# Autodesk Inventor assembly: VerticalSlides2.1
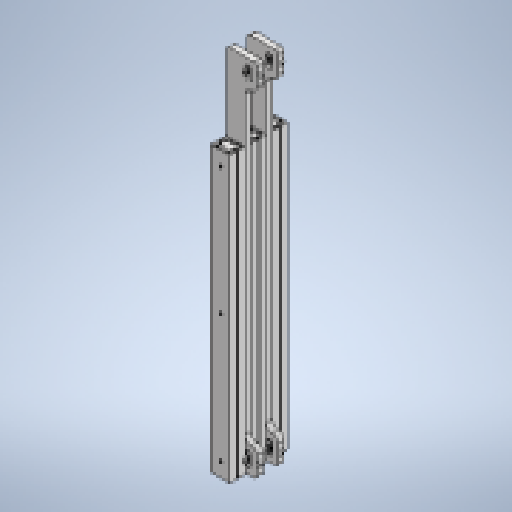
[picture p0: Inventor's stored thumbnail of the model, 512x512]
Saved by Autodesk Inventor 2023 (Build 270158000, 158)
## iProperties
Created: 2022-09-10
Part Number: VerticalSlides2.1
Document SubType Name: Assembly
Designer: deli
Author: deli
## Documents named in this file (5)
- C:\Users\deli\OneDrive - Eastside Preparatory School\FTC\8103-power-play\CAD\VerticalSlides2.1.iam
- C:\Users\deli\OneDrive - Eastside Preparatory School\FTC\8103-power-play\CAD\Middle Slide.ipt
- C:\Users\deli\OneDrive - Eastside Preparatory School\FTC\8103-power-play\CAD\FTC-parts\KC-362-30.iam
- C:\Users\deli\OneDrive - Eastside Preparatory School\FTC\8103-power-play\CAD\FTC-parts\M3\hex_socket_button_head_M3x20.ipt
- C:\Users\deli\OneDrive - Eastside Preparatory School\FTC\8103-power-play\CAD\FTC-parts\LongRobotics\3x12x4mm-bearing.ipt
## Components (7 placed, 4 different names)
1. Middle Slide:2
2. KC-362-30:2 [sub-assembly]
3. KC-362-30:3 [sub-assembly]
4. hex_socket_button_head_M3x20:2
5. hex_socket_button_head_M3x20:3
6. 3x12x4mm-bearing:1
7. 3x12x4mm-bearing:3
## Relationships (14: Mate 14)
- [Mate]: Middle Slide:2 ↔ KC-362-30:2
- [Mate]: Middle Slide:2 ↔ KC-362-30:2
- [Mate]: Middle Slide:2 ↔ KC-362-30:2
- [Mate]: Middle Slide:2 ↔ KC-362-30:3
- [Mate]: Middle Slide:2 ↔ KC-362-30:3
- [Mate]: Middle Slide:2 ↔ KC-362-30:3
- [Mate]: Middle Slide:2 ↔ hex_socket_button_head_M3x20:3
- [Mate]: Middle Slide:2 ↔ hex_socket_button_head_M3x20:2
- [Mate]: Middle Slide:2 ↔ hex_socket_button_head_M3x20:3
- [Mate]: Middle Slide:2 ↔ hex_socket_button_head_M3x20:2
- [Mate]: hex_socket_button_head_M3x20:3 ↔ 3x12x4mm-bearing:1
- [Mate] (1.175 mm): Middle Slide:2 ↔ 3x12x4mm-bearing:1
- [Mate] (1.175 mm): Middle Slide:2 ↔ 3x12x4mm-bearing:3
- [Mate]: hex_socket_button_head_M3x20:2 ↔ 3x12x4mm-bearing:3
## Named parameters: d3_d0 = 0 mm, d4_d1 = 0 mm, d5_d2 = 0 mm
